# Autodesk Inventor assembly: s-assy-shooter_frame
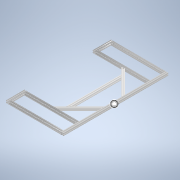
[picture p0: Inventor's stored thumbnail of the model, 180x180]
Saved by Autodesk Inventor 2022 (Build 260153000, 153)
## iProperties
Created: 2021-09-11
Part Number: s-assy-shooter_frame
Document SubType Name: Assembly
Designer: yuto6
Author: yuto6
## Documents named in this file (9)
- C:\Users\yuto6\Box\Public_Share\キャチロボバトルコンテスト2021\CAD\catchrobo_hardware\assy-shooter\s-assy-shooter_frame.iam
- C:\Users\yuto6\Box\Public_Share\キャチロボバトルコンテスト2021\CAD\catchrobo_hardware\assy-shooter\HFS5-2020-402_5.ipt
- C:\Users\yuto6\Box\Public_Share\キャチロボバトルコンテスト2021\CAD\catchrobo_hardware\assy-shooter\AIS2020_D\HPTBD5-SEP_b_.ipt
- C:\Users\yuto6\Box\Public_Share\キャチロボバトルコンテスト2021\CAD\catchrobo_hardware\assy-shooter\AIS2020_D\HNTP5-5.ipt
- C:\Users\yuto6\Box\Public_Share\キャチロボバトルコンテスト2021\CAD\catchrobo_hardware\assy-shooter\AIS2020_D\CBM5-8.ipt
- C:\Users\yuto6\Box\Public_Share\キャチロボバトルコンテスト2021\CAD\catchrobo_hardware\assy-robot\KNFS5-2020-2.ipt
- C:\Users\yuto6\Box\Public_Share\キャチロボバトルコンテスト2021\CAD\catchrobo_hardware\assy-robot\KNFS5-2020-3.ipt
- C:\Users\yuto6\Box\Public_Share\キャチロボバトルコンテスト2021\CAD\catchrobo_hardware\assy-shooter\HFBL5-2020-200.iam
- C:\Users\yuto6\Box\Public_Share\キャチロボバトルコンテスト2021\CAD\catchrobo_hardware\assy-shooter\HFBL5-2020-300.iam
## Components (20 placed, 8 different names)
1. HFS5-2020-402_5:1 — メイト:1, メイト:2, フラッシュ:1, フラッシュ:2, メイト:6, メイト:8, メイト:13, メイト:14, フラッシュ:3, フラッシュ:4, メイト:21, フラッシュ:8, メイト:24, メイト:30, フラッシュ:16
2. HFS5-2020-402_5:2 — メイト:4, メイト:5, フラッシュ:1, フラッシュ:2, メイト:6, メイト:15, メイト:16, フラッシュ:5, フラッシュ:6, メイト:22, フラッシュ:7, メイト:23, メイト:28
3. HPTBD5-SEP_b_:1 — メイト:3, メイト:7, メイト:8, メイト:9, メイト:10, メイト:11, メイト:12, メイト:19, メイト:20
4. HNTP5-5:2 — メイト:1, メイト:2, メイト:3
5. HNTP5-5:3 — メイト:4, メイト:5, メイト:7
6. CBM5-8:1 — メイト:9, メイト:11
7. CBM5-8:2 — メイト:10, メイト:12
8. HNTP5-5:4 — メイト:13, メイト:14, メイト:17
9. HNTP5-5:5 — メイト:15, メイト:16, メイト:18
10. CBM5-8:3 — メイト:17, メイト:20
11. CBM5-8:4 — メイト:18, メイト:19
12. KNFS5-2020-2:1 — フラッシュ:5, フラッシュ:6, メイト:22, フラッシュ:9, フラッシュ:10, メイト:25
13. KNFS5-2020-2:2 — フラッシュ:3, フラッシュ:4, メイト:21, フラッシュ:12, フラッシュ:13, メイト:26
14. KNFS5-2020-2:3 — フラッシュ:7, メイト:23, フラッシュ:11, フラッシュ:15, メイト:27
15. KNFS5-2020-2:4 — フラッシュ:8, メイト:24, フラッシュ:14, メイト:29
16. KNFS5-2020-3:1 — フラッシュ:9, フラッシュ:10, メイト:25, フラッシュ:11
17. KNFS5-2020-3:2 — フラッシュ:12, フラッシュ:13, メイト:26, フラッシュ:14
18. HFBL5-2020-200:1 [sub-assembly] — フラッシュ:15, メイト:27, メイト:28, メイト:32
19. HFBL5-2020-200:2 [sub-assembly] — メイト:29, メイト:30, フラッシュ:16, フラッシュ:17, メイト:31
20. HFBL5-2020-300:1 [sub-assembly] — フラッシュ:17, メイト:31, メイト:32
## Relationships (49: Mate 32, Flush 17)
- メイト:1 [Mate]: HFS5-2020-402_5:1 ↔ HNTP5-5:2
- メイト:2 [Mate]: HFS5-2020-402_5:1 ↔ HNTP5-5:2
- メイト:3 [Mate]: HPTBD5-SEP_b_:1 ↔ HNTP5-5:2
- メイト:4 [Mate]: HFS5-2020-402_5:2 ↔ HNTP5-5:3
- メイト:5 [Mate]: HFS5-2020-402_5:2 ↔ HNTP5-5:3
- フラッシュ:1 [Flush]: HFS5-2020-402_5:1 ↔ HFS5-2020-402_5:2
- フラッシュ:2 [Flush]: HFS5-2020-402_5:1 ↔ HFS5-2020-402_5:2
- メイト:6 [Mate]: HFS5-2020-402_5:1 ↔ HFS5-2020-402_5:2
- メイト:7 [Mate]: HPTBD5-SEP_b_:1 ↔ HNTP5-5:3
- メイト:8 [Mate]: HFS5-2020-402_5:1 ↔ HPTBD5-SEP_b_:1
- メイト:9 [Mate]: HPTBD5-SEP_b_:1 ↔ CBM5-8:1
- メイト:10 [Mate]: HPTBD5-SEP_b_:1 ↔ CBM5-8:2
- メイト:11 [Mate]: HPTBD5-SEP_b_:1 ↔ CBM5-8:1
- メイト:12 [Mate]: HPTBD5-SEP_b_:1 ↔ CBM5-8:2
- メイト:13 [Mate]: HFS5-2020-402_5:1 ↔ HNTP5-5:4
- メイト:14 [Mate]: HFS5-2020-402_5:1 ↔ HNTP5-5:4
- メイト:15 [Mate]: HFS5-2020-402_5:2 ↔ HNTP5-5:5
- メイト:16 [Mate]: HFS5-2020-402_5:2 ↔ HNTP5-5:5
- メイト:17 [Mate]: HNTP5-5:4 ↔ CBM5-8:3
- メイト:18 [Mate]: HNTP5-5:5 ↔ CBM5-8:4
- メイト:19 [Mate]: HPTBD5-SEP_b_:1 ↔ CBM5-8:4
- メイト:20 [Mate]: HPTBD5-SEP_b_:1 ↔ CBM5-8:3
- フラッシュ:3 [Flush]: HFS5-2020-402_5:1 ↔ KNFS5-2020-2:2
- フラッシュ:4 [Flush]: HFS5-2020-402_5:1 ↔ KNFS5-2020-2:2
- メイト:21 [Mate]: HFS5-2020-402_5:1 ↔ KNFS5-2020-2:2
- フラッシュ:5 [Flush]: HFS5-2020-402_5:2 ↔ KNFS5-2020-2:1
- フラッシュ:6 [Flush]: HFS5-2020-402_5:2 ↔ KNFS5-2020-2:1
- メイト:22 [Mate]: HFS5-2020-402_5:2 ↔ KNFS5-2020-2:1
- フラッシュ:7 [Flush]: HFS5-2020-402_5:2 ↔ KNFS5-2020-2:3
- メイト:23 [Mate]: HFS5-2020-402_5:2 ↔ KNFS5-2020-2:3
- フラッシュ:8 [Flush]: HFS5-2020-402_5:1 ↔ KNFS5-2020-2:4
- メイト:24 [Mate]: HFS5-2020-402_5:1 ↔ KNFS5-2020-2:4
- フラッシュ:9 [Flush]: KNFS5-2020-2:1 ↔ KNFS5-2020-3:1
- フラッシュ:10 [Flush]: KNFS5-2020-2:1 ↔ KNFS5-2020-3:1
- メイト:25 [Mate]: KNFS5-2020-2:1 ↔ KNFS5-2020-3:1
- フラッシュ:11 [Flush]: KNFS5-2020-2:3 ↔ KNFS5-2020-3:1
- フラッシュ:12 [Flush]: KNFS5-2020-2:2 ↔ KNFS5-2020-3:2
- フラッシュ:13 [Flush]: KNFS5-2020-2:2 ↔ KNFS5-2020-3:2
- メイト:26 [Mate]: KNFS5-2020-2:2 ↔ KNFS5-2020-3:2
- フラッシュ:14 [Flush]: KNFS5-2020-2:4 ↔ KNFS5-2020-3:2
- フラッシュ:15 [Flush]: KNFS5-2020-2:3 ↔ HFBL5-2020-200:1
- メイト:27 [Mate]: KNFS5-2020-2:3 ↔ HFBL5-2020-200:1
- メイト:28 [Mate]: HFS5-2020-402_5:2 ↔ HFBL5-2020-200:1
- メイト:29 [Mate]: KNFS5-2020-2:4 ↔ HFBL5-2020-200:2
- メイト:30 [Mate]: HFS5-2020-402_5:1 ↔ HFBL5-2020-200:2
- フラッシュ:16 [Flush]: HFS5-2020-402_5:1 ↔ HFBL5-2020-200:2
- フラッシュ:17 [Flush]: HFBL5-2020-200:2 ↔ HFBL5-2020-300:1
- メイト:31 [Mate]: HFBL5-2020-200:2 ↔ HFBL5-2020-300:1
- メイト:32 [Mate]: HFBL5-2020-200:1 ↔ HFBL5-2020-300:1
